# Autodesk Inventor assembly: Pick_&_Place_Nozzle_Assembly
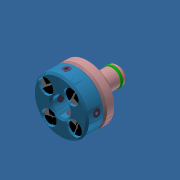
[picture p0: Inventor's stored thumbnail of the model, 180x180]
Saved by Autodesk Inventor 2015 (Build 190159000, 159)
## iProperties
Created: 2015-01-06
Part Number: Pick_&_Place_Nozzle_Assembly
Document SubType Name: Assembly
Designer: ice
Author: ice
## Documents named in this file (8)
- C:\Users\ice\Documents\GitHub\PnP-Magnetic-Tool-Tip\Inventor\Extender_Assembly_Rev_B.iam
- C:\Users\ice\Documents\GitHub\PnP-Magnetic-Tool-Tip\Inventor\Extender_Split_Top_Rev_B.ipt
- C:\Users\ice\Documents\GitHub\PnP-Magnetic-Tool-Tip\Inventor\Extender_Split_Bottom_Rev_B.ipt
- C:\Users\ice\Documents\GitHub\PnP-Magnetic-Tool-Tip\Inventor\M2x5_D963.ipt
- C:\Users\ice\Documents\GitHub\PnP-Magnetic-Tool-Tip\Inventor\o_ring_3.18_0.5.ipt
- C:\Users\ice\Documents\GitHub\PnP-Magnetic-Tool-Tip\Inventor\M2x5_Headless.ipt
- C:\Users\ice\Documents\GitHub\PnP-Magnetic-Tool-Tip\Inventor\Magnet10x1x5.ipt
- C:\Users\ice\Documents\GitHub\PnP-Magnetic-Tool-Tip\Inventor\o_ring_4.29_0.5.ipt
## Components (14 placed, 7 different names)
1. Extender_Split_Bottom_Rev_B:1 — Mate:2, Mate:4, Mate:5, Mate:6, Mate:7, Mate:8, Mate:9, Mate:10, Mate:11, Mate:22, Mate:23, Mate:29, Mate:30, Mate:31, Mate:32, Mate:33, Flush:7, Flush:8, Mate:34
2. Extender_Split_Top_Rev_B:1 — Mate:2, Mate:21, Mate:22, Mate:23, Mate:24, Mate:25, Flush:3, Mate:26, Mate:27, Flush:4, Flush:5, Mate:28, Flush:6
3. M2x5_D963:1 — Mate:4, Mate:5
4. M2x5_D963:2 — Mate:6, Mate:11
5. M2x5_D963:3 — Mate:8, Mate:9
6. M2x5_D963:4 — Mate:7, Mate:10
7. o_ring_3.18_0.5:1 — Mate:24, Mate:25
8. Magnet10x1x5:1 — Mate:21, Flush:3
9. o_ring_4.29_0.5:1 — Mate:27, Flush:4
10. o_ring_4.29_0.5:2 — Mate:26, Flush:5
11. M2x5_Headless:1 — Mate:32, Mate:33
12. M2x5_Headless:2 — Mate:30, Mate:34
13. M2x5_Headless:3 — Mate:31, Flush:7
14. M2x5_Headless:4 — Mate:29, Flush:8
## Relationships (29: Mate 23, Flush 6)
- Mate:2: Extender_Split_Bottom_Rev_B:1 ↔ Extender_Split_Top_Rev_B:1
- Mate:4: Extender_Split_Bottom_Rev_B:1 ↔ M2x5_D963:1
- Mate:5: Extender_Split_Bottom_Rev_B:1 ↔ M2x5_D963:1
- Mate:6: Extender_Split_Bottom_Rev_B:1 ↔ M2x5_D963:2
- Mate:7: Extender_Split_Bottom_Rev_B:1 ↔ M2x5_D963:4
- Mate:8: Extender_Split_Bottom_Rev_B:1 ↔ M2x5_D963:3
- Mate:9: Extender_Split_Bottom_Rev_B:1 ↔ M2x5_D963:3
- Mate:10: Extender_Split_Bottom_Rev_B:1 ↔ M2x5_D963:4
- Mate:11: Extender_Split_Bottom_Rev_B:1 ↔ M2x5_D963:2
- Mate:21: Extender_Split_Top_Rev_B:1 ↔ Magnet10x1x5:1
- Mate:22: Extender_Split_Bottom_Rev_B:1 ↔ Extender_Split_Top_Rev_B:1
- Mate:23: Extender_Split_Bottom_Rev_B:1 ↔ Extender_Split_Top_Rev_B:1
- Mate:24: Extender_Split_Top_Rev_B:1 ↔ o_ring_3.18_0.5:1
- Mate:25: Extender_Split_Top_Rev_B:1 ↔ o_ring_3.18_0.5:1
- Flush:3: Extender_Split_Top_Rev_B:1 ↔ Magnet10x1x5:1
- Mate:26: Extender_Split_Top_Rev_B:1 ↔ o_ring_4.29_0.5:2
- Mate:27: Extender_Split_Top_Rev_B:1 ↔ o_ring_4.29_0.5:1
- Flush:4: Extender_Split_Top_Rev_B:1 ↔ o_ring_4.29_0.5:1
- Flush:5: Extender_Split_Top_Rev_B:1 ↔ o_ring_4.29_0.5:2
- Mate:28: Extender_Split_Top_Rev_B:1
- Flush:6: Extender_Split_Top_Rev_B:1
- Mate:29: Extender_Split_Bottom_Rev_B:1 ↔ M2x5_Headless:4
- Mate:30: Extender_Split_Bottom_Rev_B:1 ↔ M2x5_Headless:2
- Mate:31: Extender_Split_Bottom_Rev_B:1 ↔ M2x5_Headless:3
- Mate:32: Extender_Split_Bottom_Rev_B:1 ↔ M2x5_Headless:1
- Mate:33: Extender_Split_Bottom_Rev_B:1 ↔ M2x5_Headless:1
- Flush:7: Extender_Split_Bottom_Rev_B:1 ↔ M2x5_Headless:3
- Flush:8: Extender_Split_Bottom_Rev_B:1 ↔ M2x5_Headless:4
- Mate:34: Extender_Split_Bottom_Rev_B:1 ↔ M2x5_Headless:2
